# Autodesk Inventor assembly: Assembly1
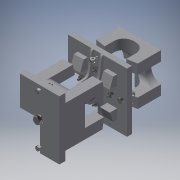
[picture p0: Inventor's stored thumbnail of the model, 180x180]
Saved by Autodesk Inventor 2019 (Build 230136000, 136)
## iProperties
Created: 2018-06-02
Part Number: Assembly1
Document SubType Name: Assembly
Designer: Till
Mass: 914.286 g
Surface Area: 1989.21 cm^2
Volume: 819.475 cm^3
Density: 1.1157 g/cm^3
Author: Till
## Documents named in this file (14)
- D:\Dokuments_HDD\Inventor\HumRob\Draft1_Ankle\Assembly1.iam
- D:\Dokuments_HDD\Inventor\HumRob\Draft1_Ankle\KBRM_12_1.iam
- D:\Dokuments_HDD\Inventor\HumRob\Draft1_Ankle\GBM_12_1.ipt
- D:\Dokuments_HDD\Inventor\HumRob\Draft1_Ankle\WFM_1214_04_3.ipt
- D:\Dokuments_HDD\Inventor\HumRob\Draft1_Ankle\DoubleFork_lower.ipt
- C:\Users\Till\Documents\Inventor\Content Center Files\R2019\en-US\GB 798-88\Eye bolt GB 798 M5 x 25.ipt
- C:\Users\Till\Documents\Inventor\Content Center Files\R2019\en-US\ANSI B18.2.4.2M\ANSI B18.2.4.2M - M5x0,8 - 8.ipt
- D:\Dokuments_HDD\Inventor\HumRob\Draft1_Ankle\Foot_Ankl_Connector.ipt
- C:\Users\Till\Documents\Inventor\Content Center Files\R2019\en-US\DIN 433-1  A\DIN 433 - 8,4.ipt
- C:\Users\Till\Documents\Inventor\Content Center Files\R2019\en-US\DIN EN 24 017\ISO 4017 - M8 x 70DIN EN.ipt
- D:\Dokuments_HDD\Inventor\HumRob\Draft1_Ankle\Leg_Adapter.ipt
- C:\Users\Till\Documents\Inventor\Content Center Files\R2019\en-US\DIN EN 24 017\ISO 4017 - M4 x 20DIN EN.ipt
- C:\Users\Till\Documents\Inventor\Content Center Files\R2019\en-US\DIN 988(1)\DIN 988 - S9 x 15.ipt
- C:\Users\Till\Documents\Inventor\Content Center Files\R2019\en-US\DIN EN 24 017\ISO 4017 - M8 x 25DIN EN.ipt
## Components (38 placed, 13 different names)
1. KBRM_12_1:1 [sub-assembly] — Mate:1, Mate:2, Mate:7, Mate:9, Mate:20, Angle:3, Mate:46, Mate:47, Mate:48, Mate:79, Mate:81
2. GBM_12_1:1 — Mate:9, Mate:23
3. WFM_1214_04_3:1 — Mate:21
4. WFM_1214_04_3:2 — Mate:7, Mate:22
5. Fork:1 — Mate:12, Mate:13, Mate:14, Mate:15, Mate:18, Angle:2, Mate:24, Mate:25, Mate:26, Mate:27, Angle:4, Angle:5, Mate:51, Mate:52, Mate:53, Mate:54, Mate:55, Mate:56, Mate:57, Mate:58, Mate:59, Mate:60, Mate:62
6. Fork:2 — Mate:20, Mate:21, Mate:22, Mate:23, Mate:24, Angle:3, Mate:25, Mate:26, Mate:29, Mate:30, Mate:32, Mate:49, Mate:50, Angle:8, Angle:9, Mate:63, Mate:64, Mate:65, Mate:66, Mate:67, Mate:68, Mate:71, Mate:72, Mate:73, Mate:74, Mate:77, Mate:78
7. KBRM_12_1:2 [sub-assembly] — Mate:16, Mate:17, Mate:19, Angle:2, Mate:33, Mate:34, Mate:35, Mate:42
8. WFM_1214_04_3:3 — Mate:14, Mate:15, Mate:17
9. WFM_1214_04_3:4 — Mate:12, Mate:13, Mate:16
10. GBM_12_1:2 — Mate:18, Mate:19
11. Bolt GB/T 798-1988 M5 x 25:1 — Mate:27, Mate:28, Flush:1, Angle:4
12. ANSI B18.2.4.2M M5x0,8:1 — Mate:28, Mate:29, Flush:1
13. Bolt GB/T 798-1988 M5 x 25:2 — Mate:30, Mate:31, Flush:2, Angle:5
14. ANSI B18.2.4.2M M5x0,8:2 — Mate:31, Mate:32, Flush:2
15. Foot_Ankl_Connector:1 — Mate:33, Mate:34, Mate:35, Mate:36, Angle:6, Mate:37, Angle:7, Mate:39, Mate:41, Mate:44
16. Bolt GB/T 798-1988 M5 x 25:3 — Mate:36, Angle:6, Mate:38, Flush:3
17. Bolt GB/T 798-1988 M5 x 25:4 — Mate:37, Angle:7, Mate:40, Flush:4
18. ANSI B18.2.4.2M M5x0,8:3 — Mate:38, Mate:39, Flush:3
19. ANSI B18.2.4.2M M5x0,8:4 — Mate:40, Mate:41, Flush:4
20. DIN EN 24017 M8 x 70:1 — Mate:42, Mate:43, Mate:45
21. DIN 433-1 A 8,4:1 — Mate:43, Mate:44, Mate:45
22. Leg_Adapter:1 — Mate:46, Mate:47, Mate:48, Mate:80
23. Bolt GB/T 798-1988 M5 x 25:5 — Mate:50, Mate:61, Flush:5, Angle:9
24. Bolt GB/T 798-1988 M5 x 25:6 — Mate:49, Flush:6, Angle:8
25. ANSI B18.2.4.2M M5x0,8:5 — Mate:51, Mate:62, Flush:6
26. ANSI B18.2.4.2M M5x0,8:6 — Mate:55, Mate:59
27. ANSI B18.2.4.2M M5x0,8:7 — Mate:54, Mate:58
28. ANSI B18.2.4.2M M5x0,8:8 — Mate:53, Mate:57
29. ANSI B18.2.4.2M M5x0,8:9 — Mate:52, Mate:56
30. ANSI B18.2.4.2M M5x0,8:10 — Mate:60, Mate:61, Flush:5
31. DIN EN 24017 M4 x 20:1 — Mate:63, Mate:64
32. DIN EN 24017 M4 x 20:2 — Mate:65, Mate:66
33. DIN EN 24017 M4 x 20:3 — Mate:67, Mate:68
34. DIN EN 24017 M4 x 20:5 — Mate:71, Mate:72
35. DIN EN 24017 M4 x 20:6 — Mate:73, Mate:74
36. DIN EN 24017 M4 x 20:8 — Mate:77, Mate:78
37. DIN 988 S9 x 15:1 — Mate:79, Mate:80, Mate:82
38. DIN EN 24017 M8 x 25:1 — Mate:81, Mate:82
## Relationships (85: Mate 71, Angle 8, Flush 6)
- Mate:1: KBRM_12_1:1
- Mate:2: KBRM_12_1:1
- Mate:7: KBRM_12_1:1 ↔ WFM_1214_04_3:2
- Mate:9: KBRM_12_1:1 ↔ GBM_12_1:1
- Mate:12: Fork:1 ↔ WFM_1214_04_3:4
- Mate:13: Fork:1 ↔ WFM_1214_04_3:4
- Mate:14: Fork:1 ↔ WFM_1214_04_3:3
- Mate:15: Fork:1 ↔ WFM_1214_04_3:3
- Mate:16: KBRM_12_1:2 ↔ WFM_1214_04_3:4
- Mate:17: KBRM_12_1:2 ↔ WFM_1214_04_3:3
- Mate:18: Fork:1 ↔ GBM_12_1:2
- Mate:19: KBRM_12_1:2 ↔ GBM_12_1:2
- Angle:2 (180 deg): Fork:1 ↔ KBRM_12_1:2
- Mate:20: KBRM_12_1:1 ↔ Fork:2
- Mate:21: WFM_1214_04_3:1 ↔ Fork:2
- Mate:22: WFM_1214_04_3:2 ↔ Fork:2
- Mate:23: GBM_12_1:1 ↔ Fork:2
- Mate:24: Fork:1 ↔ Fork:2
- Angle:3 (0 deg): KBRM_12_1:1 ↔ Fork:2
- Mate:25: Fork:1 ↔ Fork:2
- Mate:26: Fork:1 ↔ Fork:2
- Mate:27: Fork:1 ↔ Bolt GB/T 798-1988 M5 x 25:1
- Mate:28: Bolt GB/T 798-1988 M5 x 25:1 ↔ ANSI B18.2.4.2M M5x0,8:1
- Mate:29: Fork:2 ↔ ANSI B18.2.4.2M M5x0,8:1
- Flush:1: Bolt GB/T 798-1988 M5 x 25:1 ↔ ANSI B18.2.4.2M M5x0,8:1
- Angle:4 (0 deg): Fork:1 ↔ Bolt GB/T 798-1988 M5 x 25:1
- Mate:30: Fork:2 ↔ Bolt GB/T 798-1988 M5 x 25:2
- Mate:31: Bolt GB/T 798-1988 M5 x 25:2 ↔ ANSI B18.2.4.2M M5x0,8:2
- Mate:32: Fork:2 ↔ ANSI B18.2.4.2M M5x0,8:2
- Flush:2: Bolt GB/T 798-1988 M5 x 25:2 ↔ ANSI B18.2.4.2M M5x0,8:2
- Angle:5 (0 deg): Fork:1 ↔ Bolt GB/T 798-1988 M5 x 25:2
- Mate:33: KBRM_12_1:2 ↔ Foot_Ankl_Connector:1
- Mate:34: KBRM_12_1:2 ↔ Foot_Ankl_Connector:1
- Mate:35: KBRM_12_1:2 ↔ Foot_Ankl_Connector:1
- Mate:36: Foot_Ankl_Connector:1 ↔ Bolt GB/T 798-1988 M5 x 25:3
- Angle:6 (0 deg): Foot_Ankl_Connector:1 ↔ Bolt GB/T 798-1988 M5 x 25:3
- Mate:37: Foot_Ankl_Connector:1 ↔ Bolt GB/T 798-1988 M5 x 25:4
- Angle:7 (0 deg): Foot_Ankl_Connector:1 ↔ Bolt GB/T 798-1988 M5 x 25:4
- Mate:38: Bolt GB/T 798-1988 M5 x 25:3 ↔ ANSI B18.2.4.2M M5x0,8:3
- Mate:39: Foot_Ankl_Connector:1 ↔ ANSI B18.2.4.2M M5x0,8:3
- Flush:3: Bolt GB/T 798-1988 M5 x 25:3 ↔ ANSI B18.2.4.2M M5x0,8:3
- Mate:40: Bolt GB/T 798-1988 M5 x 25:4 ↔ ANSI B18.2.4.2M M5x0,8:4
- Mate:41: Foot_Ankl_Connector:1 ↔ ANSI B18.2.4.2M M5x0,8:4
- Flush:4: Bolt GB/T 798-1988 M5 x 25:4 ↔ ANSI B18.2.4.2M M5x0,8:4
- Mate:42: KBRM_12_1:2 ↔ DIN EN 24017 M8 x 70:1
- Mate:43: DIN EN 24017 M8 x 70:1 ↔ DIN 433-1 A 8,4:1
- Mate:44: Foot_Ankl_Connector:1 ↔ DIN 433-1 A 8,4:1
- Mate:45: DIN EN 24017 M8 x 70:1 ↔ DIN 433-1 A 8,4:1
- Mate:46: KBRM_12_1:1 ↔ Leg_Adapter:1
- Mate:47: KBRM_12_1:1 ↔ Leg_Adapter:1
- Mate:48: KBRM_12_1:1 ↔ Leg_Adapter:1
- Mate:49: Fork:2 ↔ Bolt GB/T 798-1988 M5 x 25:6
- Mate:50: Fork:2 ↔ Bolt GB/T 798-1988 M5 x 25:5
- Mate:51: Fork:1 ↔ ANSI B18.2.4.2M M5x0,8:5
- Mate:52: Fork:1 ↔ ANSI B18.2.4.2M M5x0,8:9
- Mate:53: Fork:1 ↔ ANSI B18.2.4.2M M5x0,8:8
- Mate:54: Fork:1 ↔ ANSI B18.2.4.2M M5x0,8:7
- Mate:55: Fork:1 ↔ ANSI B18.2.4.2M M5x0,8:6
- Mate:56: Fork:1 ↔ ANSI B18.2.4.2M M5x0,8:9
- Mate:57: Fork:1 ↔ ANSI B18.2.4.2M M5x0,8:8
- Mate:58: Fork:1 ↔ ANSI B18.2.4.2M M5x0,8:7
- Mate:59: Fork:1 ↔ ANSI B18.2.4.2M M5x0,8:6
- Mate:60: Fork:1 ↔ ANSI B18.2.4.2M M5x0,8:10
- Mate:61: Bolt GB/T 798-1988 M5 x 25:5 ↔ ANSI B18.2.4.2M M5x0,8:10
- Flush:5: Bolt GB/T 798-1988 M5 x 25:5 ↔ ANSI B18.2.4.2M M5x0,8:10
- Mate:62: Fork:1 ↔ ANSI B18.2.4.2M M5x0,8:5
- Flush:6: Bolt GB/T 798-1988 M5 x 25:6 ↔ ANSI B18.2.4.2M M5x0,8:5
- Angle:8 (0 deg): Fork:2 ↔ Bolt GB/T 798-1988 M5 x 25:6
- Angle:9 (0 deg): Fork:2 ↔ Bolt GB/T 798-1988 M5 x 25:5
- Mate:63: Fork:2 ↔ DIN EN 24017 M4 x 20:1
- Mate:64: Fork:2 ↔ DIN EN 24017 M4 x 20:1
- Mate:65: Fork:2 ↔ DIN EN 24017 M4 x 20:2
- Mate:66: Fork:2 ↔ DIN EN 24017 M4 x 20:2
- Mate:67: Fork:2 ↔ DIN EN 24017 M4 x 20:3
- Mate:68: Fork:2 ↔ DIN EN 24017 M4 x 20:3
- Mate:71: Fork:2 ↔ DIN EN 24017 M4 x 20:5
- Mate:72: Fork:2 ↔ DIN EN 24017 M4 x 20:5
- Mate:73: Fork:2 ↔ DIN EN 24017 M4 x 20:6
- Mate:74: Fork:2 ↔ DIN EN 24017 M4 x 20:6
- Mate:77: Fork:2 ↔ DIN EN 24017 M4 x 20:8
- Mate:78: Fork:2 ↔ DIN EN 24017 M4 x 20:8
- Mate:79: KBRM_12_1:1 ↔ DIN 988 S9 x 15:1
- Mate:80: Leg_Adapter:1 ↔ DIN 988 S9 x 15:1
- Mate:81: KBRM_12_1:1 ↔ DIN EN 24017 M8 x 25:1
- Mate:82: DIN 988 S9 x 15:1 ↔ DIN EN 24017 M8 x 25:1
## Named parameters: roll_angle = 180 deg, pitch_angle = 0 deg
